# Autodesk Inventor assembly: Infinity_holders
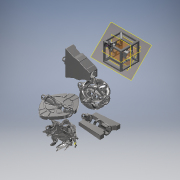
[picture p0: Inventor's stored thumbnail of the model, 180x180]
Saved by Autodesk Inventor 2019 (Build 230136000, 136)
## iProperties
Created: 2019-05-18
Part Number: Infinity_holders
Document SubType Name: Assembly
Designer: Jorian Brusind
Author: Jorian Brusind
## Documents named in this file (7)
- C:\Users\Jorian Brusind\Documents\GitHub\PersonalProjects\Inventor Projects\Infinity\Infinity_holders.iam
- C:\Users\Jorian Brusind\Documents\GitHub\PersonalProjects\Inventor Projects\Infinity\Waves.ipt
- C:\Users\Jorian Brusind\Documents\GitHub\PersonalProjects\Inventor Projects\Infinity\Spires.ipt
- C:\Users\Jorian Brusind\Documents\GitHub\PersonalProjects\Inventor Projects\Infinity\Orb.ipt
- C:\Users\Jorian Brusind\Documents\GitHub\PersonalProjects\Inventor Projects\Infinity\Inner.ipt
- C:\Users\Jorian Brusind\Documents\GitHub\PersonalProjects\Inventor Projects\Infinity\Holder.ipt
- C:\Users\Jorian Brusind\Documents\GitHub\PersonalProjects\Inventor Projects\Infinity\Agamoto.ipt
## Components (6 placed, 6 different names)
1. Waves:1 — Flush:5
2. Spires:1 — Flush:4
3. Orb:1 — Flush:3
4. Inner:1 — Flush:1
5. Holder:1 — Flush:1, Flush:2, Flush:3, Flush:4, Flush:5
6. Agamoto:1 — Flush:2
## Relationships (5: Flush 5)
- Flush:1: Inner:1 ↔ Holder:1
- Flush:2: Holder:1 ↔ Agamoto:1
- Flush:3: Orb:1 ↔ Holder:1
- Flush:4: Spires:1 ↔ Holder:1
- Flush:5: Waves:1 ↔ Holder:1
